# Autodesk Inventor assembly: mesoSPIM_xyzr_stages
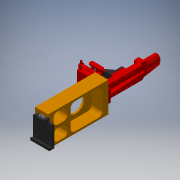
[picture p0: Inventor's stored thumbnail of the model, 180x180]
Saved by Autodesk Inventor 2016 (Build 200138000, 138)
## iProperties
Created: 2018-08-27
Part Number: mesoSPIM_xyzr_stages
Document SubType Name: Assembly
Designer: voigt
Author: voigt
## Documents named in this file (6)
- D:\Microscope_Design\CAD_Files\mesoSPIM_design\mesoSPIM\sample_stages\mesoSPIM_xyzr_stages.iam
- D:\Microscope_Design\CAD_Files\mesoSPIM_design\library\Thorlabs\X95_accessoires\XT95P11_M.ipt
- D:\Microscope_Design\CAD_Files\mesoSPIM_design\mesoSPIM\sample_stages\birdhouse.ipt
- D:\Microscope_Design\CAD_Files\mesoSPIM_design\library\Physik_Instrumente\Aufbau_DYNEOS_mesoSPIM.ipt
- D:\Microscope_Design\CAD_Files\mesoSPIM_design\mesoSPIM\sample_stages\M-116-Adapter.ipt
- D:\Microscope_Design\CAD_Files\mesoSPIM_design\library\Thorlabs\posts\post_mounts\PH20_M.ipt
## Components (5 placed, 5 different names)
1. XT95P11_M:1 — Mate:1, Mate:2, Angle:1
2. birdhouse:1 — Mate:1, Mate:2, Angle:1, Mate:3, Mate:4, Mate:5
3. Aufbau_DYNEOS_mesoSPIM:1 — Mate:3, Mate:4, Mate:5, Mate:6, Mate:7
4. M-116-Adapter:1 — Mate:6, Mate:7, Mate:8, Mate:9
5. PH20_M:1 — Mate:8, Mate:9
## Relationships (10: Mate 9, Angle 1)
- Mate:1: XT95P11_M:1 ↔ birdhouse:1
- Mate:2: XT95P11_M:1 ↔ birdhouse:1
- Angle:1 (0 deg): XT95P11_M:1 ↔ birdhouse:1
- Mate:3: birdhouse:1 ↔ Aufbau_DYNEOS_mesoSPIM:1
- Mate:4: birdhouse:1 ↔ Aufbau_DYNEOS_mesoSPIM:1
- Mate:5: birdhouse:1 ↔ Aufbau_DYNEOS_mesoSPIM:1
- Mate:6: Aufbau_DYNEOS_mesoSPIM:1 ↔ M-116-Adapter:1
- Mate:7: Aufbau_DYNEOS_mesoSPIM:1 ↔ M-116-Adapter:1
- Mate:8: M-116-Adapter:1 ↔ PH20_M:1
- Mate:9: M-116-Adapter:1 ↔ PH20_M:1
